# Autodesk Inventor assembly: Złożenie ramienia robota
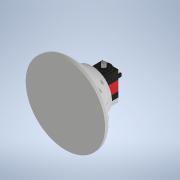
[picture p0: Inventor's stored thumbnail of the model, 180x180]
Saved by Autodesk Inventor 2021 (Build 250183000, 183)
## iProperties
Created: 2021-11-03
Part Number: Złożenie ramienia robota
Document SubType Name: Assembly
Designer: Łukasz
Author: Łukasz
## Documents named in this file (6)
- E:\GITHUB_Czołg\Szybki-Czolg-antyRadziecki\Ramie robota\Ramie robota\Złożenie ramienia robota.iam
- E:\GITHUB_Czołg\Szybki-Czolg-antyRadziecki\Ramie robota\Ramie robota\Podstawa 01-1.ipt
- E:\GITHUB_Czołg\Szybki-Czolg-antyRadziecki\Ramie robota\Ramie robota\Podstawa 01-2.ipt
- E:\GITHUB_Czołg\Szybki-Czolg-antyRadziecki\Ramie robota\Ramie robota\serwo 30x70.ipt
- E:\GITHUB_Czołg\Szybki-Czolg-antyRadziecki\Ramie robota\Ramie robota\mocowanie lozyska 10-1.ipt
- C:\Users\Łukasz\Documents\Inventor\Content Center Files\R2021\en-US\BS 292 (I)\BS 292 Part 1 - 608 - 8 x 22 x 7.ipt
## Components (5 placed, 5 different names)
1. Podstawa 01-1:1 — Mate:1, Mate:2, Mate:3
2. Podstawa 01-2:1 — Mate:4, Mate:5, Mate:6
3. serwo 30x70:1 — Mate:1, Mate:2, Mate:3, Mate:4, Mate:5, Mate:6, Mate:7, Flush:1, Flush:2
4. mocowanie lozyska 10-1:1 — Mate:7, Flush:1, Flush:2, Rotational:1
5. BS 292: Part 1 (I) (Metric) 608 - 8 x 22 x 7:1 — Rotational:1
## Relationships (10: Mate 7, Flush 2, RevoluteJoint 1)
- Mate:1: Podstawa 01-1:1 ↔ serwo 30x70:1
- Mate:2: Podstawa 01-1:1 ↔ serwo 30x70:1
- Mate:3: Podstawa 01-1:1 ↔ serwo 30x70:1
- Mate:4: Podstawa 01-2:1 ↔ serwo 30x70:1
- Mate:5: Podstawa 01-2:1 ↔ serwo 30x70:1
- Mate:6: Podstawa 01-2:1 ↔ serwo 30x70:1
- Mate:7: serwo 30x70:1 ↔ mocowanie lozyska 10-1:1
- Flush:1: serwo 30x70:1 ↔ mocowanie lozyska 10-1:1
- Flush:2: serwo 30x70:1 ↔ mocowanie lozyska 10-1:1
- Rotational:1 [RevoluteJoint]: mocowanie lozyska 10-1:1 ↔ BS 292: Part 1 (I) (Metric) 608 - 8 x 22 x 7:1
